# Autodesk Inventor assembly: Main
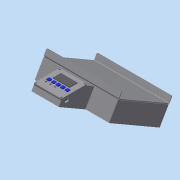
[picture p0: Inventor's stored thumbnail of the model, 180x180]
Saved by Autodesk Inventor 2018 (Build 220112000, 112)
## iProperties
Created: 2020-10-03
Part Number: Main
Material: Generisch
Document SubType Name: Assembly
Designer: marce
Author: marce
## Documents named in this file (10)
- C:\Users\marce\Documents\Waage\CAD\Main.iam
- C:\Users\marce\Documents\Waage\CAD\PCB\PCB.iam
- C:\Users\marce\Documents\Waage\CAD\Schiled.ipt
- C:\Users\marce\Documents\Waage\CAD\Taster.ipt
- C:\Users\marce\Documents\Waage\CAD\Gehause.ipt
- C:\Users\marce\Documents\Waage\CAD\Unterlagscheibe.ipt
- C:\Users\marce\Documents\Waage\CAD\LCD_Distanz.ipt
- C:\Users\marce\Documents\Waage\CAD\Hauptplatte.ipt
- C:\Users\marce\Documents\Waage\CAD\LoadCell.ipt
- C:\Users\marce\Documents\Waage\CAD\Schale.ipt
## Components (21 placed, 9 different names)
1. PCB:1 [sub-assembly] — Passend:1, Passend:2, Passend:3, Passend:18, Passend:26, Passend:27, Passend:28, Passend:37, Passend:38, Passend:39, Passend:40, Passend:41, Passend:42, Passend:43, Passend:44, Passend:45
2. Schiled:1 — Passend:1, Passend:2, Passend:3, Passend:4, Passend:7, Passend:12, Passend:14, Passend:16, Passend:17, Passend:19, Fluchtend:1, Passend:20, Passend:29, Passend:30, Passend:31, Passend:32, Passend:33, Passend:34, Passend:35, Passend:36
3. Taster:1 — Passend:16, Passend:32, Passend:33
4. Taster:2 — Passend:4, Passend:18, Passend:36
5. Taster:3 — Passend:7, Passend:17, Passend:34, Passend:35
6. Taster:4 — Passend:29, Passend:30, Passend:45
7. Taster:5 — Passend:12, Passend:14, Passend:31
8. Gehause:1 — Passend:19, Fluchtend:1, Passend:20, Passend:21, Passend:22, Passend:23, Passend:24, Passend:25, Passend:46, Fluchtend:4, Fluchtend:5
9. Unterlagscheibe:1 — Passend:23, Passend:26
10. Unterlagscheibe:2 — Passend:24, Passend:25
11. Unterlagscheibe:3 — Passend:22, Passend:27
12. Unterlagscheibe:4 — Passend:21, Passend:28
13. LCD_Distanz:1 — Passend:42, Passend:43
14. LCD_Distanz:2 — Passend:41, Passend:44
15. LCD_Distanz:3 — Passend:37, Passend:40
16. LCD_Distanz:4 — Passend:38, Passend:39
17. Hauptplatte:1 — Passend:46, Fluchtend:4, Fluchtend:5, Passend:47, Passend:48, Passend:49, Passend:50, Passend:51, Passend:52, Passend:53, Passend:54, Passend:55, Fluchtend:6, Fluchtend:7
18. LoadCell:1 — Passend:47, Passend:48, Passend:49
19. LoadCell:2 — Passend:50, Passend:54, Passend:55
20. LoadCell:3 — Passend:51, Passend:52, Passend:53, Passend:56
21. Schale:1 — Passend:56, Fluchtend:6, Fluchtend:7
## Relationships (53: Mate 48, Flush 5)
- Passend:1 [Mate] (3.5 mm): PCB:1 ↔ Schiled:1
- Passend:2 [Mate]: PCB:1 ↔ Schiled:1
- Passend:3 [Mate]: PCB:1 ↔ Schiled:1
- Passend:4 [Mate]: Schiled:1 ↔ Taster:2
- Passend:7 [Mate]: Schiled:1 ↔ Taster:3
- Passend:12 [Mate]: Schiled:1 ↔ Taster:5
- Passend:14 [Mate]: Schiled:1 ↔ Taster:5
- Passend:16 [Mate]: Schiled:1 ↔ Taster:1
- Passend:17 [Mate]: Schiled:1 ↔ Taster:3
- Passend:18 [Mate]: PCB:1 ↔ Taster:2
- Passend:19 [Mate]: Schiled:1 ↔ Gehause:1
- Fluchtend:1 [Flush]: Schiled:1 ↔ Gehause:1
- Passend:20 [Mate]: Schiled:1 ↔ Gehause:1
- Passend:21 [Mate]: Gehause:1 ↔ Unterlagscheibe:4
- Passend:22 [Mate]: Gehause:1 ↔ Unterlagscheibe:3
- Passend:23 [Mate]: Gehause:1 ↔ Unterlagscheibe:1
- Passend:24 [Mate]: Gehause:1 ↔ Unterlagscheibe:2
- Passend:25 [Mate]: Gehause:1 ↔ Unterlagscheibe:2
- Passend:26 [Mate]: PCB:1 ↔ Unterlagscheibe:1
- Passend:27 [Mate]: PCB:1 ↔ Unterlagscheibe:3
- Passend:28 [Mate]: PCB:1 ↔ Unterlagscheibe:4
- Passend:29 [Mate]: Schiled:1 ↔ Taster:4
- Passend:30 [Mate]: Schiled:1 ↔ Taster:4
- Passend:31 [Mate]: Schiled:1 ↔ Taster:5
- Passend:32 [Mate]: Schiled:1 ↔ Taster:1
- Passend:33 [Mate]: Schiled:1 ↔ Taster:1
- Passend:34 [Mate]: Schiled:1 ↔ Taster:3
- Passend:35 [Mate]: Schiled:1 ↔ Taster:3
- Passend:36 [Mate]: Schiled:1 ↔ Taster:2
- Passend:37 [Mate]: PCB:1 ↔ LCD_Distanz:3
- Passend:38 [Mate]: PCB:1 ↔ LCD_Distanz:4
- Passend:39 [Mate]: PCB:1 ↔ LCD_Distanz:4
- Passend:40 [Mate]: PCB:1 ↔ LCD_Distanz:3
- Passend:41 [Mate]: PCB:1 ↔ LCD_Distanz:2
- Passend:42 [Mate]: PCB:1 ↔ LCD_Distanz:1
- Passend:43 [Mate]: PCB:1 ↔ LCD_Distanz:1
- Passend:44 [Mate]: PCB:1 ↔ LCD_Distanz:2
- Passend:45 [Mate]: PCB:1 ↔ Taster:4
- Passend:46 [Mate]: Gehause:1 ↔ Hauptplatte:1
- Fluchtend:4 [Flush]: Gehause:1 ↔ Hauptplatte:1
- Fluchtend:5 [Flush] (-72.5 mm): Gehause:1 ↔ Hauptplatte:1
- Passend:47 [Mate]: Hauptplatte:1 ↔ LoadCell:1
- Passend:48 [Mate]: Hauptplatte:1 ↔ LoadCell:1
- Passend:49 [Mate]: Hauptplatte:1 ↔ LoadCell:1
- Passend:50 [Mate]: Hauptplatte:1 ↔ LoadCell:2
- Passend:51 [Mate]: Hauptplatte:1 ↔ LoadCell:3
- Passend:52 [Mate]: Hauptplatte:1 ↔ LoadCell:3
- Passend:53 [Mate]: Hauptplatte:1 ↔ LoadCell:3
- Passend:54 [Mate]: Hauptplatte:1 ↔ LoadCell:2
- Passend:55 [Mate]: Hauptplatte:1 ↔ LoadCell:2
- Passend:56 [Mate] (2 mm): LoadCell:3 ↔ Schale:1
- Fluchtend:6 [Flush]: Hauptplatte:1 ↔ Schale:1
- Fluchtend:7 [Flush]: Hauptplatte:1 ↔ Schale:1
